# Autodesk Inventor assembly: Assembly
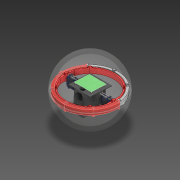
[picture p0: Inventor's stored thumbnail of the model, 180x180]
Saved by Autodesk Inventor 2022 (Build 260153000, 153)
## iProperties
Created: 2022-03-04
Part Number: Assembly
Document SubType Name: Assembly
Designer: 32497
Author: 32497
## Documents named in this file (24)
- D:\Users\Seppe\Documents\OneDrive\OneDrive - Vrije Universiteit Brussel\VUB\3 BAIW\Bachelorproef\Shared Folder\CAD\CAD\V7\Assembly.iam
- D:\Users\Seppe\Documents\OneDrive\OneDrive - Vrije Universiteit Brussel\VUB\3 BAIW\Bachelorproef\Shared Folder\CAD\CAD\V7\BoardDrager.ipt
- D:\Users\Seppe\Documents\OneDrive\OneDrive - Vrije Universiteit Brussel\VUB\3 BAIW\Bachelorproef\Shared Folder\CAD\CAD\V7\servo.ipt
- D:\Users\Seppe\Documents\OneDrive\OneDrive - Vrije Universiteit Brussel\VUB\3 BAIW\Bachelorproef\Shared Folder\CAD\CAD\V7\Bol.ipt
- D:\Users\Seppe\Documents\OneDrive\OneDrive - Vrije Universiteit Brussel\VUB\3 BAIW\Bachelorproef\Shared Folder\CAD\CAD\V7\Moer_4.ipt
- D:\Users\Seppe\Documents\OneDrive\OneDrive - Vrije Universiteit Brussel\VUB\3 BAIW\Bachelorproef\Shared Folder\CAD\CAD\V7\standoff.ipt
- D:\Users\Seppe\Documents\OneDrive\OneDrive - Vrije Universiteit Brussel\VUB\3 BAIW\Bachelorproef\Shared Folder\CAD\CAD\V7\Batterij_Groot.ipt
- D:\Users\Seppe\Documents\OneDrive\OneDrive - Vrije Universiteit Brussel\VUB\3 BAIW\Bachelorproef\Shared Folder\CAD\CAD\V7\Batterij_Klein.ipt
- D:\Users\Seppe\Documents\OneDrive\OneDrive - Vrije Universiteit Brussel\VUB\3 BAIW\Bachelorproef\Shared Folder\CAD\CAD\V7\M25x3 Bolt.ipt
- D:\Users\Seppe\Documents\OneDrive\OneDrive - Vrije Universiteit Brussel\VUB\3 BAIW\Bachelorproef\Shared Folder\CAD\CAD\V7\61901 Bearing.ipt
- D:\Users\Seppe\Documents\OneDrive\OneDrive - Vrije Universiteit Brussel\VUB\3 BAIW\Bachelorproef\Shared Folder\CAD\CAD\V7\BinnenringMiddenStuk.ipt
- D:\Users\Seppe\Documents\OneDrive\OneDrive - Vrije Universiteit Brussel\VUB\3 BAIW\Bachelorproef\Shared Folder\CAD\CAD\V7\BinnenringStuk1.ipt
- D:\Users\Seppe\Documents\OneDrive\OneDrive - Vrije Universiteit Brussel\VUB\3 BAIW\Bachelorproef\Shared Folder\CAD\CAD\V7\BinnenringStuk2.ipt
- D:\Users\Seppe\Documents\OneDrive\OneDrive - Vrije Universiteit Brussel\VUB\3 BAIW\Bachelorproef\Shared Folder\CAD\CAD\V7\Ring_Gear1.iam
- D:\Users\Seppe\Documents\OneDrive\OneDrive - Vrije Universiteit Brussel\VUB\3 BAIW\Bachelorproef\Shared Folder\CAD\CAD\V7\Ring_Gear2.iam
- D:\Users\Seppe\Documents\OneDrive\OneDrive - Vrije Universiteit Brussel\VUB\3 BAIW\Bachelorproef\Shared Folder\CAD\CAD\V7\Ring_Gear3.iam
- D:\Users\Seppe\Documents\OneDrive\OneDrive - Vrije Universiteit Brussel\VUB\3 BAIW\Bachelorproef\Shared Folder\CAD\CAD\V7\Ring_Gear4.iam
- D:\Users\Seppe\Documents\OneDrive\OneDrive - Vrije Universiteit Brussel\VUB\3 BAIW\Bachelorproef\Shared Folder\CAD\CAD\V7\Ring_Gear5.iam
- D:\Users\Seppe\Documents\OneDrive\OneDrive - Vrije Universiteit Brussel\VUB\3 BAIW\Bachelorproef\Shared Folder\CAD\CAD\V7\Ring_Gear6.iam
- D:\Users\Seppe\Documents\OneDrive\OneDrive - Vrije Universiteit Brussel\VUB\3 BAIW\Bachelorproef\Shared Folder\CAD\CAD\V7\Ring_Gear7.iam
- D:\Users\Seppe\Documents\OneDrive\OneDrive - Vrije Universiteit Brussel\VUB\3 BAIW\Bachelorproef\Shared Folder\CAD\CAD\V7\Ring_Gear8.iam
- D:\Users\Seppe\Documents\OneDrive\OneDrive - Vrije Universiteit Brussel\VUB\3 BAIW\Bachelorproef\Shared Folder\CAD\CAD\V7\BaarThread.ipt
- D:\Users\Seppe\Documents\OneDrive\OneDrive - Vrije Universiteit Brussel\VUB\3 BAIW\Bachelorproef\Shared Folder\CAD\CAD\V7\GearKlein.iam
- D:\Users\Seppe\Documents\OneDrive\OneDrive - Vrije Universiteit Brussel\VUB\3 BAIW\Bachelorproef\Shared Folder\CAD\CAD\V7\ProtoBoardV1.iam
## Components (52 placed, 23 different names)
1. Bol:1 — Mate:169, Mate:170, Flush:34, Mate:260
2. Bol:2 — Mate:259, Mate:260, Mate:261
3. ProtoBoardV1:1 [sub-assembly] — Mate:272, Mate:273
4. standoff:1 — Flush:50, Mate:263
5. standoff:2 — Flush:50, Flush:51, Mate:264
6. standoff:3 — Flush:51, Flush:52, Mate:262, Mate:266, Mate:272, Mate:273
7. standoff:4 — Flush:52, Mate:265
8. Moer_4:1 — Flush:37, Flush:38, Mate:239
9. Moer_4:2 — Flush:37, Mate:236, Mate:248, Mate:249
10. Moer_4:3 — Flush:38, Flush:39, Mate:242
11. Moer_4:4 — Flush:39, Mate:245
12. Moer_4:5 — Flush:40, Mate:236, Mate:237, Mate:252
13. Moer_4:6 — Flush:40, Flush:41, Mate:239, Mate:240, Mate:253
14. Moer_4:7 — Flush:41, Flush:42, Mate:242, Mate:243, Mate:255
15. Moer_4:8 — Flush:42, Mate:245, Mate:246, Mate:254
16. Moer_4:9 — Flush:43, Mate:237, Mate:238, Mate:250
17. Moer_4:10 — Flush:43, Flush:44, Mate:240, Mate:241
18. Moer_4:11 — Flush:44, Flush:45, Mate:243, Mate:244
19. Moer_4:12 — Flush:45, Mate:246, Mate:247
20. Moer_4:13 — Flush:46, Mate:238, Flush:49, Mate:251
21. Moer_4:14 — Flush:46, Flush:47, Flush:49, Mate:241
22. Moer_4:15 — Flush:47, Flush:48, Mate:244
23. Moer_4:16 — Flush:48, Mate:247
24. Ring_Gear4:1 [sub-assembly] — Mate:221, Mate:222, Mate:223
25. Ring_Gear5:1 [sub-assembly] — Mate:225, Mate:226, Mate:228, Mate:231, Mate:270, Mate:271
26. Ring_Gear1:1 [sub-assembly] — Flush:21, Mate:124, Mate:145, Mate:146, Flush:23, Mate:165, Mate:175
27. Ring_Gear2:1 [sub-assembly] — Mate:144, Mate:145, Mate:146, Flush:23, Flush:24, Mate:169, Mate:170, Mate:173, Mate:259
28. Ring_Gear3:1 [sub-assembly] — Mate:126, Mate:144, Flush:24, Tangent:1, Mate:221, Mate:222, Mate:223, Rotation:4
29. Ring_Gear6:1 [sub-assembly] — Mate:171, Mate:175, Mate:224, Mate:225, Mate:226, Mate:227, Mate:229, Mate:230
30. Ring_Gear7:1 [sub-assembly] — Mate:113, Mate:114, Flush:18, Mate:130, Mate:224
31. Ring_Gear8:1 [sub-assembly] — Mate:113, Mate:114, Flush:18, Flush:21, Mate:131, Mate:165, Mate:232
32. 61901 Bearing:2 — Flush:25, Mate:176, Mate:206, Mate:209
33. 61901 Bearing:1 — Flush:26, Mate:177, Mate:210
34. BinnenringMiddenStuk:1 — Mate:202, Mate:203, Mate:204, Mate:205, Mate:207, Mate:208, Mate:211, Mate:212
35. BinnenringStuk1:1 — Mate:202, Mate:203, Mate:206, Mate:207, Mate:209, Mate:211, Flush:33, Mate:220
36. BinnenringStuk2:1 — Mate:213, Mate:214, Mate:215, Mate:219, Flush:33, Mate:220
37. BinnenringMiddenStuk:2 — Mate:213, Mate:214, Mate:215, Mate:216, Mate:217, Mate:218
38. BinnenringStuk1:2 — Mate:204, Mate:205, Mate:208, Mate:210
39. BinnenringStuk2:2 — Mate:216, Mate:217, Mate:218
40. servo:1 — Mate:178, Mate:179, Mate:182, Mate:184, Rotation:3, Mate:185, Mate:186, Mate:251, Mate:252
41. servo:2 — Mate:180, Mate:181, Mate:183, Flush:27, Mate:188, Mate:249, Mate:250
42. GearKlein:2 [sub-assembly] — Mate:171, Mate:172, Rotation:2, Flush:25, Mate:176, Mate:178, Mate:179, Rotation:3, Rotation:4, Mate:235, Flush:36
43. GearKlein:1 [sub-assembly] — Mate:172, Mate:173, Mate:174, Tangent:1, Rotation:2, Flush:26, Mate:177, Mate:180, Mate:181, Mate:234, Flush:35
44. M25x3 Bolt:2 — Mate:235, Flush:36
45. M25x3 Bolt:1 — Mate:234, Flush:35
46. BaarThread:1 — Flush:28, Flush:29, Flush:30, Mate:186, Mate:255
47. BaarThread:2 — Flush:30, Mate:184, Mate:253
48. BaarThread:3 — Flush:29, Mate:185, Mate:189, Mate:254
49. BaarThread:4 — Mate:182, Mate:183, Flush:27, Flush:28, Mate:187, Mate:248
50. Batterij_Klein:1 — Mate:192, Mate:193, Flush:32
51. BoardDrager:1 — Mate:187, Mate:188, Mate:189, Mate:190, Mate:191, Flush:31, Mate:192, Mate:193, Flush:32, Mate:262, Mate:263, Mate:264, Mate:265, Mate:266
52. Batterij_Groot:1 — Mate:190, Mate:191, Flush:31
## Relationships (136: Mate 100, Flush 32, RelateRotation 3, Tangent 1)
- Mate:113: Ring_Gear7:1 ↔ Ring_Gear8:1
- Mate:114: Ring_Gear7:1 ↔ Ring_Gear8:1
- Flush:18: Ring_Gear7:1 ↔ Ring_Gear8:1
- Flush:21: Ring_Gear1:1 ↔ Ring_Gear8:1
- Mate:124: Ring_Gear1:1
- Mate:126: Ring_Gear3:1
- Mate:130: Ring_Gear7:1
- Mate:131: Ring_Gear8:1
- Mate:144: Ring_Gear2:1 ↔ Ring_Gear3:1
- Mate:145: Ring_Gear1:1 ↔ Ring_Gear2:1
- Mate:146: Ring_Gear1:1 ↔ Ring_Gear2:1
- Flush:23: Ring_Gear1:1 ↔ Ring_Gear2:1
- Flush:24: Ring_Gear2:1 ↔ Ring_Gear3:1
- Mate:165: Ring_Gear1:1 ↔ Ring_Gear8:1
- Mate:169: Bol:1 ↔ Ring_Gear2:1
- Mate:170: Bol:1 ↔ Ring_Gear2:1
- Mate:171: Ring_Gear6:1 ↔ GearKlein:2
- Mate:172: GearKlein:2 ↔ GearKlein:1
- Mate:173: Ring_Gear2:1 ↔ GearKlein:1
- Mate:174: GearKlein:1
- Tangent:1: Ring_Gear3:1 ↔ GearKlein:1
- Mate:175: Ring_Gear1:1 ↔ Ring_Gear6:1
- Rotation:2 [RelateRotation] (1 ul): GearKlein:2 ↔ GearKlein:1
- Flush:25: 61901 Bearing:2 ↔ GearKlein:2
- Mate:176: 61901 Bearing:2 ↔ GearKlein:2
- Flush:26: 61901 Bearing:1 ↔ GearKlein:1
- Mate:177: 61901 Bearing:1 ↔ GearKlein:1
- Mate:178: servo:1 ↔ GearKlein:2
- Mate:179: servo:1 ↔ GearKlein:2
- Mate:180: servo:2 ↔ GearKlein:1
- Mate:181: servo:2 ↔ GearKlein:1
- Mate:182: servo:1 ↔ BaarThread:4
- Mate:183: servo:2 ↔ BaarThread:4
- Flush:27 (-8.8 mm): servo:2 ↔ BaarThread:4
- Flush:28: BaarThread:1 ↔ BaarThread:4
- Flush:29: BaarThread:1 ↔ BaarThread:3
- Flush:30: BaarThread:1 ↔ BaarThread:2
- Mate:184: servo:1 ↔ BaarThread:2
- Rotation:3 [RelateRotation] (1 ul): servo:1 ↔ GearKlein:2
- Mate:185: servo:1 ↔ BaarThread:3
- Mate:186: servo:1 ↔ BaarThread:1
- Mate:187: BaarThread:4 ↔ BoardDrager:1
- Mate:188 (15 mm): servo:2 ↔ BoardDrager:1
- Mate:189: BaarThread:3 ↔ BoardDrager:1
- Mate:190: BoardDrager:1 ↔ Batterij_Groot:1
- Mate:191: BoardDrager:1 ↔ Batterij_Groot:1
- Flush:31: BoardDrager:1 ↔ Batterij_Groot:1
- Mate:192: Batterij_Klein:1 ↔ BoardDrager:1
- Mate:193: Batterij_Klein:1 ↔ BoardDrager:1
- Flush:32: Batterij_Klein:1 ↔ BoardDrager:1
- Mate:202: BinnenringMiddenStuk:1 ↔ BinnenringStuk1:1
- Mate:203: BinnenringMiddenStuk:1 ↔ BinnenringStuk1:1
- Mate:204: BinnenringMiddenStuk:1 ↔ BinnenringStuk1:2
- Mate:205: BinnenringMiddenStuk:1 ↔ BinnenringStuk1:2
- Mate:206: 61901 Bearing:2 ↔ BinnenringStuk1:1
- Mate:207: BinnenringMiddenStuk:1 ↔ BinnenringStuk1:1
- Mate:208: BinnenringMiddenStuk:1 ↔ BinnenringStuk1:2
- Mate:209: 61901 Bearing:2 ↔ BinnenringStuk1:1
- Mate:210: 61901 Bearing:1 ↔ BinnenringStuk1:2
- Mate:211: BinnenringMiddenStuk:1 ↔ BinnenringStuk1:1
- Mate:212: BinnenringMiddenStuk:1
- Mate:213: BinnenringStuk2:1 ↔ BinnenringMiddenStuk:2
- Mate:214: BinnenringStuk2:1 ↔ BinnenringMiddenStuk:2
- Mate:215: BinnenringStuk2:1 ↔ BinnenringMiddenStuk:2
- Mate:216: BinnenringMiddenStuk:2 ↔ BinnenringStuk2:2
- Mate:217: BinnenringMiddenStuk:2 ↔ BinnenringStuk2:2
- Mate:218: BinnenringMiddenStuk:2 ↔ BinnenringStuk2:2
- Mate:219: BinnenringStuk2:1
- Flush:33: BinnenringStuk1:1 ↔ BinnenringStuk2:1
- Mate:220: BinnenringStuk1:1 ↔ BinnenringStuk2:1
- Mate:221: Ring_Gear4:1 ↔ Ring_Gear3:1
- Mate:222: Ring_Gear4:1 ↔ Ring_Gear3:1
- Mate:223: Ring_Gear4:1 ↔ Ring_Gear3:1
- Mate:224: Ring_Gear6:1 ↔ Ring_Gear7:1
- Mate:225: Ring_Gear5:1 ↔ Ring_Gear6:1
- Mate:226: Ring_Gear5:1 ↔ Ring_Gear6:1
- Mate:227: Ring_Gear6:1
- Mate:228: Ring_Gear5:1
- Mate:229: Ring_Gear6:1
- Mate:230: Ring_Gear6:1
- Mate:231: Ring_Gear5:1
- Mate:232: Ring_Gear8:1
- Flush:34: Bol:1
- Rotation:4 [RelateRotation] (0.059 ul): Ring_Gear3:1 ↔ GearKlein:2
- Mate:234: GearKlein:1 ↔ M25x3 Bolt:1
- Flush:35 (-5 mm): GearKlein:1 ↔ M25x3 Bolt:1
- Mate:235: GearKlein:2 ↔ M25x3 Bolt:2
- Flush:36 (-5 mm): GearKlein:2 ↔ M25x3 Bolt:2
- Flush:37: Moer_4:1 ↔ Moer_4:2
- Flush:38: Moer_4:1 ↔ Moer_4:3
- Flush:39: Moer_4:3 ↔ Moer_4:4
- Flush:40: Moer_4:5 ↔ Moer_4:6
- Flush:41: Moer_4:6 ↔ Moer_4:7
- Flush:42: Moer_4:7 ↔ Moer_4:8
- Flush:43: Moer_4:9 ↔ Moer_4:10
- Flush:44: Moer_4:10 ↔ Moer_4:11
- Flush:45: Moer_4:11 ↔ Moer_4:12
- Flush:46: Moer_4:13 ↔ Moer_4:14
- Flush:47: Moer_4:14 ↔ Moer_4:15
- Flush:48: Moer_4:15 ↔ Moer_4:16
- Mate:236: Moer_4:2 ↔ Moer_4:5
- Mate:237: Moer_4:5 ↔ Moer_4:9
- Mate:238: Moer_4:9 ↔ Moer_4:13
- Flush:49: Moer_4:13 ↔ Moer_4:14
- Mate:239: Moer_4:1 ↔ Moer_4:6
- Mate:240: Moer_4:6 ↔ Moer_4:10
- Mate:241: Moer_4:10 ↔ Moer_4:14
- Mate:242: Moer_4:3 ↔ Moer_4:7
- Mate:243: Moer_4:7 ↔ Moer_4:11
- Mate:244: Moer_4:11 ↔ Moer_4:15
- Mate:245: Moer_4:4 ↔ Moer_4:8
- Mate:246: Moer_4:8 ↔ Moer_4:12
- Mate:247: Moer_4:12 ↔ Moer_4:16
- Mate:248: Moer_4:2 ↔ BaarThread:4
- Mate:249: Moer_4:2 ↔ servo:2
- Mate:250: Moer_4:9 ↔ servo:2
- Mate:251: Moer_4:13 ↔ servo:1
- Mate:252: Moer_4:5 ↔ servo:1
- Mate:253: Moer_4:6 ↔ BaarThread:2
- Mate:254: Moer_4:8 ↔ BaarThread:3
- Mate:255: Moer_4:7 ↔ BaarThread:1
- Mate:259: Bol:2 ↔ Ring_Gear2:1
- Mate:260: Bol:1 ↔ Bol:2
- Mate:261: Bol:2
- Flush:50: standoff:1 ↔ standoff:2
- Flush:51: standoff:2 ↔ standoff:3
- Flush:52: standoff:3 ↔ standoff:4
- Mate:262: standoff:3 ↔ BoardDrager:1
- Mate:263: standoff:1 ↔ BoardDrager:1
- Mate:264: standoff:2 ↔ BoardDrager:1
- Mate:265: standoff:4 ↔ BoardDrager:1
- Mate:266: standoff:3 ↔ BoardDrager:1
- Mate:270: Ring_Gear5:1
- Mate:271: Ring_Gear5:1
- Mate:272: ProtoBoardV1:1 ↔ standoff:3
- Mate:273: ProtoBoardV1:1 ↔ standoff:3
